# Autodesk Inventor assembly: part_assembly
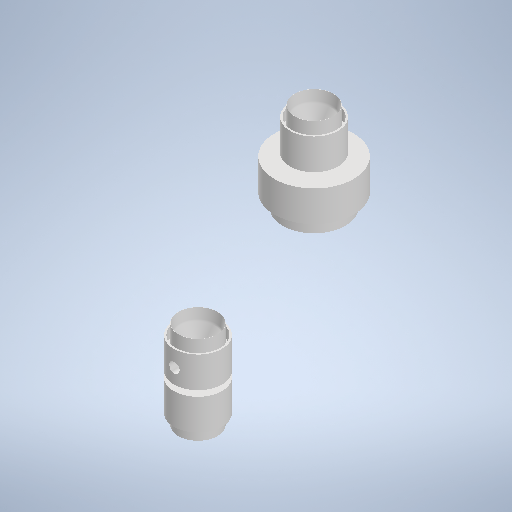
[picture p0: Inventor's stored thumbnail of the model, 512x512]
Saved by Autodesk Inventor 2025 (Build 290162010, 162A)
## iProperties
Created: 2023-05-02
Part Number: part_assembly
Document SubType Name: Assembly
Designer: dinesh
Author: dinesh
## Documents named in this file (4)
- C:\Users\dinesh\Documents\GitHub\flytools\flyporter\adapter\flyport_adapter_assemblies.iam
- C:\Users\dinesh\Documents\GitHub\flytools\flyporter\adapter\flyport_adapter.ipt
- C:\Users\dinesh\Documents\GitHub\flytools\flyporter\vial\flyport_vial.ipt
- C:\Users\dinesh\Documents\GitHub\flytools\flyporter\bottle\flyport_bottle.ipt
## Components (6 placed, 3 different names)
1. flyport_adapter:1 — Mate:1, Mate:2, Mate:3
2. flyport_vial:1 — Mate:1, Mate:2
3. flyport_vial:2 — Mate:3
4. flyport_bottle:1 — Mate:4, Mate:5
5. flyport_vial:3 — Mate:6
6. flyport_adapter:2 — Mate:4, Mate:5, Mate:6
## Relationships (6: Mate 6)
- Mate:1: flyport_adapter:1 ↔ flyport_vial:1
- Mate:2: flyport_adapter:1 ↔ flyport_vial:1
- Mate:3: flyport_adapter:1 ↔ flyport_vial:2
- Mate:4: flyport_bottle:1 ↔ flyport_adapter:2
- Mate:5: flyport_bottle:1 ↔ flyport_adapter:2
- Mate:6: flyport_vial:3 ↔ flyport_adapter:2
